# Autodesk Inventor assembly: Makitronics-FaceShield-V1
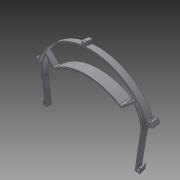
[picture p0: Inventor's stored thumbnail of the model, 180x180]
Saved by Autodesk Inventor 2015 (Build 190159000, 159)
## iProperties
Created: 2020-03-25
Part Number: Makitronics-FaceShield-V1
Document SubType Name: Assembly
Designer: Dominick Lee
Author: Dominick Lee
## Documents named in this file (3)
- C:\Users\Dominick\Documents\GitHub\COVID19-Prevention-Tools\Makitronics Face Shield\Makitronics-FaceShield-V1.iam
- C:\Users\Dominick\Documents\GitHub\COVID19-Prevention-Tools\Makitronics Face Shield\Makitronics-FaceShield.ipt
- C:\Users\Dominick\Documents\GitHub\COVID19-Prevention-Tools\Makitronics Face Shield\BagClip.ipt
## Components (4 placed, 2 different names)
1. Makitronics-FaceShield:1 — Rigid:1, Rigid:2, Rigid:3
2. BagClip:1 — Rigid:1
3. BagClip:2 — Rigid:2
4. BagClip:3 — Rigid:3
## Relationships (3: WeldJoint 3)
- Rigid:1 [WeldJoint]: Makitronics-FaceShield:1 ↔ BagClip:1
- Rigid:2 [WeldJoint]: Makitronics-FaceShield:1 ↔ BagClip:2
- Rigid:3 [WeldJoint]: Makitronics-FaceShield:1 ↔ BagClip:3
